# Autodesk Inventor assembly: 12-26 Full V2
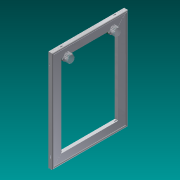
[picture p0: Inventor's stored thumbnail of the model, 180x180]
Saved by Autodesk Inventor 2013 (Build 170138000, 138)
## iProperties
Created: 2013-08-18
Part Number: 12-26 Full V2
Document SubType Name: Assembly
Designer: Sawaiz
Author: Sawaiz
## Documents named in this file (3)
- S:\Sawaiz\Documents\3D Modeling\Inventor\PolarGraph\12-26 Full V2.iam
- S:\Sawaiz\Documents\3D Modeling\Inventor\PolarGraph\12-16 Frame.iam
- S:\Sawaiz\Documents\3D Modeling\Inventor\PolarGraph\MotorAssemblyV4.iam
## Components (3 placed, 2 different names)
1. 12-16 Frame:1 [sub-assembly] — Mate:1, Mate:2, Mate:3, Mate:4, Mate:5, Mate:6
2. MotorAssemblyV4:1 [sub-assembly] — Mate:1, Mate:4, Mate:6
3. MotorAssemblyV4:2 [sub-assembly] — Mate:2, Mate:3, Mate:5
## Relationships (6: Mate 6)
- Mate:1: 12-16 Frame:1 ↔ MotorAssemblyV4:1
- Mate:2: 12-16 Frame:1 ↔ MotorAssemblyV4:2
- Mate:3: 12-16 Frame:1 ↔ MotorAssemblyV4:2
- Mate:4: 12-16 Frame:1 ↔ MotorAssemblyV4:1
- Mate:5: 12-16 Frame:1 ↔ MotorAssemblyV4:2
- Mate:6: 12-16 Frame:1 ↔ MotorAssemblyV4:1
